# Autodesk Inventor assembly: Robot!
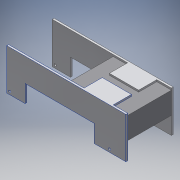
[picture p0: Inventor's stored thumbnail of the model, 180x180]
Saved by Autodesk Inventor 2016 (Build 200138000, 138)
## iProperties
Created: 2015-10-31
Part Number: Robot!
Document SubType Name: Assembly
Designer: rossmosier
Author: rossmosier
## Documents named in this file (4)
- C:\Users\rossmosier\Documents\CAD Team\CADTeam\Assemblies\Robot!.iam
- C:\Users\rossmosier\Documents\CAD Team\CADTeam\Parts\Brain.ipt
- C:\Users\rossmosier\Documents\CAD Team\CADTeam\Drive Train\Side.ipt
- C:\Users\rossmosier\Documents\CAD Team\CADTeam\Drive Train\rightSide.ipt
## Components (3 placed, 3 different names)
1. Brain:1 — Mate:1, Mate:2
2. Side:1 — Mate:2
3. rightSide:1 — Mate:1
## Relationships (2: Mate 2)
- Mate:1: Brain:1 ↔ rightSide:1
- Mate:2: Brain:1 ↔ Side:1
